# Autodesk Inventor assembly: Moving Carousel Section Assembly
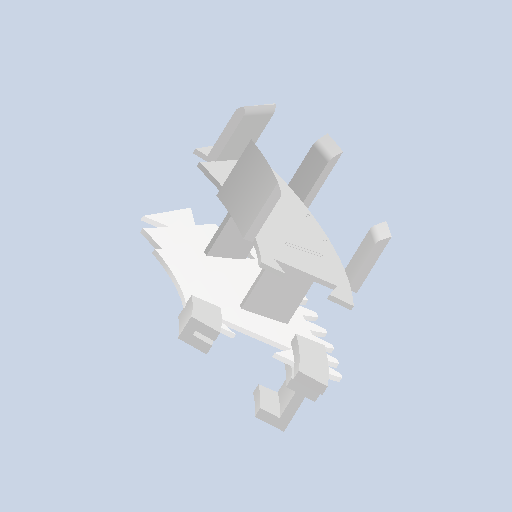
[picture p0: Inventor's stored thumbnail of the model, 512x512]
Saved by Autodesk Inventor 2023 (Build 270158000, 158)
## iProperties
Created: 2023-02-14
Part Number: Moving Carousel Section Assembly
Document SubType Name: Assembly
Designer: cheng
Author: cheng
## Documents named in this file (6)
- C:\Users\mihal\Desktop\12a th Assembly\Moving Carousel\Moving Carousel Section Assembly.iam
- C:\Users\mihal\Desktop\12a th Assembly\Moving Carousel\Moving Caoursel Base.ipt
- C:\Users\mihal\Desktop\12a th Assembly\Moving Carousel\Moving Carousel Wall.ipt
- C:\Users\mihal\Desktop\12a th Assembly\Moving Carousel\Moving Caoursel base Clip.ipt
- C:\Users\mihal\Desktop\12a th Assembly\Moving Carousel\Moving Carousel Base Inner Clip.ipt
- C:\Users\mihal\Desktop\12a th Assembly\Moving Carousel\Moving Carousel Upper.ipt
## Components (7 placed, 5 different names)
1. Moving Carousel Wall:1 — Mate:3, Flush:2, Mate:4
2. Moving Carousel Wall:2 — Flush:3, Mate:5, Mate:6, Mate:13, Flush:4, Mate:14
3. Moving Carousel Wall:3 — Flush:1, Mate:1, Mate:2
4. Moving Caoursel Base:1 — Flush:1, Mate:1, Mate:2, Mate:3, Flush:2, Mate:4, Flush:3, Mate:5, Mate:6, Mate:7, Mate:8, Mate:9, Mate:10, Mate:11, Mate:12
5. Moving Caoursel base Clip:1 — Mate:7, Mate:8, Mate:9
6. Moving Carousel Base Inner Clip:1 — Mate:10, Mate:11, Mate:12
7. Moving Carousel Upper:1 — Mate:13, Flush:4, Mate:14
## Relationships (18: Mate 14, Flush 4)
- Flush:1: Moving Carousel Wall:3 ↔ Moving Caoursel Base:1
- Mate:1: Moving Carousel Wall:3 ↔ Moving Caoursel Base:1
- Mate:2: Moving Carousel Wall:3 ↔ Moving Caoursel Base:1
- Mate:3: Moving Carousel Wall:1 ↔ Moving Caoursel Base:1
- Flush:2: Moving Carousel Wall:1 ↔ Moving Caoursel Base:1
- Mate:4: Moving Carousel Wall:1 ↔ Moving Caoursel Base:1
- Flush:3: Moving Carousel Wall:2 ↔ Moving Caoursel Base:1
- Mate:5: Moving Carousel Wall:2 ↔ Moving Caoursel Base:1
- Mate:6: Moving Carousel Wall:2 ↔ Moving Caoursel Base:1
- Mate:7: Moving Caoursel Base:1 ↔ Moving Caoursel base Clip:1
- Mate:8: Moving Caoursel Base:1 ↔ Moving Caoursel base Clip:1
- Mate:9: Moving Caoursel Base:1 ↔ Moving Caoursel base Clip:1
- Mate:10: Moving Caoursel Base:1 ↔ Moving Carousel Base Inner Clip:1
- Mate:11: Moving Caoursel Base:1 ↔ Moving Carousel Base Inner Clip:1
- Mate:12: Moving Caoursel Base:1 ↔ Moving Carousel Base Inner Clip:1
- Mate:13: Moving Carousel Wall:2 ↔ Moving Carousel Upper:1
- Flush:4: Moving Carousel Wall:2 ↔ Moving Carousel Upper:1
- Mate:14: Moving Carousel Wall:2 ↔ Moving Carousel Upper:1
